# Autodesk Inventor assembly: Baugruppe1
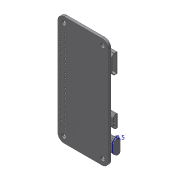
[picture p0: Inventor's stored thumbnail of the model, 180x180]
Saved by Autodesk Inventor 2021.3 (Build 253353000, 353)
## iProperties
Company: Schneeberger Lineartechnik AG
RuleStatus: InUse
Created: 2021-09-28
Part Number: Baugruppe1
User Status: Schnelländerung
Document SubType Name: Assembly
Designer: SRORF
Mass: 3.30931 g
Surface Area: 58.5832 cm^2
Volume: 3.30931 cm^3
Density: 1 g/cm^3
Author: SRORF
Status: Produktion Freigegeben
ROT_Density: 0.0
PDB_Ident_Ver: =<PDB_Ident> <PDB_Version>
ROT_Weight: 0.003 kg
ROT_Weight_Num: 0.0033093086390339967
## Documents named in this file (3)
- C:\kt\WorkSpace\Uhr\CAD\Baugruppe1.iam
- C:\kt\WorkSpace\Uhr\CAD\RaspberryPiZeroW.ipt
- C:\kt\WorkSpace\Uhr\CAD\Power_Cap.ipt
## Components (2 placed, 2 different names)
1. RaspberryPiZeroW:1 — Fluchtend:1, Passend:1, Passend:2, Passend:3
2. Power_Cap:1 — Passend:1, Passend:2, Passend:3
## Relationships (4: Mate 3, Flush 1)
- Fluchtend:1 [Flush]: RaspberryPiZeroW:1
- Passend:1 [Mate]: RaspberryPiZeroW:1 ↔ Power_Cap:1
- Passend:2 [Mate]: RaspberryPiZeroW:1 ↔ Power_Cap:1
- Passend:3 [Mate]: RaspberryPiZeroW:1 ↔ Power_Cap:1
